# Autodesk Inventor assembly: robot_frame
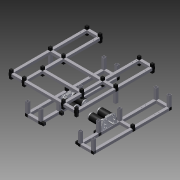
[picture p0: Inventor's stored thumbnail of the model, 180x180]
Saved by Autodesk Inventor 2011 SP1 (Build 150282100, 282)
## iProperties
Created: 2013-01-17
Part Number: robot_frame
Document SubType Name: Assembly
Designer: Christopher
Author: Christopher
## Documents named in this file (4)
- \\WW427-DATA1\StuHome\971065\Documents\GitHub\Robotics 2112 Yes 2112\2013CAD\2013 robot\Spiderbot\robot_frame.iam
- \\WW427-DATA1\StuHome\971065\Documents\GitHub\Robotics 2112 Yes 2112\2013CAD\2013 robot\forklift\robot parts\robot_frame_layer1.iam
- \\WW427-DATA1\StuHome\971065\Documents\GitHub\Robotics 2112 Yes 2112\2013CAD\2013 robot\forklift\robot parts\1tube_4_midlayer.ipt
- \\WW427-DATA1\StuHome\971065\Documents\GitHub\Robotics 2112 Yes 2112\2013CAD\2013 robot\forklift\robot parts\robot_frame_layer2.iam
## Components (16 placed, 3 different names)
1. robot_frame_layer1:1 [sub-assembly]
2. 1tube_4_midlayer:1
3. 1tube_4_midlayer:2
4. 1tube_4_midlayer:3 — Mate:4, Mate:5, Mate:6
5. 1tube_4_midlayer:4
6. 1tube_4_midlayer:5
7. 1tube_4_midlayer:6
8. 1tube_4_midlayer:7 — Mate:1, Mate:2, Mate:3
9. 1tube_4_midlayer:8
10. 1tube_4_midlayer:9
11. 1tube_4_midlayer:10
12. 1tube_4_midlayer:11
13. 1tube_4_midlayer:12
14. 1tube_4_midlayer:13
15. 1tube_4_midlayer:14
16. robot_frame_layer2:1 [sub-assembly] — Mate:1, Mate:2, Mate:3, Mate:4, Mate:5, Mate:6
## Relationships (6: Mate 6)
- Mate:1: 1tube_4_midlayer:7 ↔ robot_frame_layer2:1
- Mate:2: 1tube_4_midlayer:7 ↔ robot_frame_layer2:1
- Mate:3: 1tube_4_midlayer:7 ↔ robot_frame_layer2:1
- Mate:4: 1tube_4_midlayer:3 ↔ robot_frame_layer2:1
- Mate:5: 1tube_4_midlayer:3 ↔ robot_frame_layer2:1
- Mate:6: 1tube_4_midlayer:3 ↔ robot_frame_layer2:1
